# Autodesk Inventor assembly: Final Assembly
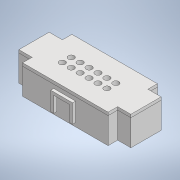
[picture p0: Inventor's stored thumbnail of the model, 180x180]
Saved by Autodesk Inventor 2021 (Build 250183000, 183)
## iProperties
Created: 2020-11-23
Part Number: Final Assembly
Document SubType Name: Assembly
Designer: coupe
Mass: 176.766 g
Surface Area: 1412.79 cm^2
Volume: 176.766 cm^3
Density: 1 g/cm^3
Author: coupe
## Documents named in this file (5)
- C:\Users\coupe\OneDrive\Desktop\ENGINEER 1P13\Design Studios\P2\Container Design\Assembly FInal.iam
- C:\Users\coupe\OneDrive\Desktop\ENGINEER 1P13\Design Studios\P2\Container Design\Container Final.ipt
- C:\Users\coupe\OneDrive\Desktop\ENGINEER 1P13\Design Studios\P2\Autodesk Inventor\Surgical Tools\Tweezer.ipt
- C:\Users\coupe\OneDrive\Desktop\ENGINEER 1P13\Design Studios\P2\Container Design\Lid Final.ipt
- C:\Users\coupe\OneDrive\Desktop\ENGINEER 1P13\Design Studios\P2\Container Design\Footprint.ipt
## Components (4 placed, 4 different names)
1. Container Final:1 — Flush:1, Flush:2, Flush:3, Transitional:1, Mate:5, Transitional:2, Mate:6, Mate:7, Mate:8, Angle:1, Angle:2, Mate:9, Mate:10, Mate:11
2. Tweezer:1 — Transitional:1, Mate:5, Transitional:2, Angle:1, Angle:2
3. Lid Final:1 — Mate:6, Mate:7, Mate:8
4. Footprint:1 — Mate:9, Mate:10, Mate:11
## Relationships (14: Mate 7, Flush 3, Transitional 2, Angle 2)
- Flush:1: Container Final:1
- Flush:2: Container Final:1
- Flush:3: Container Final:1
- Transitional:1: Container Final:1 ↔ Tweezer:1
- Mate:5 (0.95 mm): Container Final:1 ↔ Tweezer:1
- Transitional:2: Container Final:1 ↔ Tweezer:1
- Mate:6: Container Final:1 ↔ Lid Final:1
- Mate:7: Container Final:1 ↔ Lid Final:1
- Mate:8: Container Final:1 ↔ Lid Final:1
- Angle:1 (180 deg): Container Final:1 ↔ Tweezer:1
- Angle:2 (176.32 deg): Container Final:1 ↔ Tweezer:1
- Mate:9: Container Final:1 ↔ Footprint:1
- Mate:10: Container Final:1 ↔ Footprint:1
- Mate:11: Container Final:1 ↔ Footprint:1
